# Autodesk Inventor assembly: Odom_Assembly_II
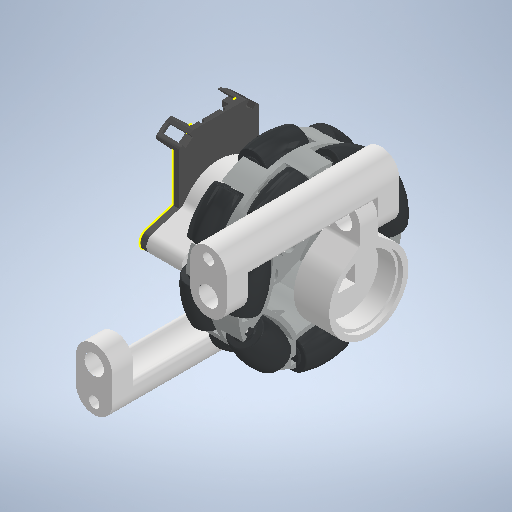
[picture p0: Inventor's stored thumbnail of the model, 512x512]
Saved by Autodesk Inventor 2025.1 (Build 291241020, 241B)
## iProperties
Created: 2024-11-16
Part Number: Odom_Assembly_II
Document SubType Name: Assembly
Designer: AtuStem
Author: AtuStem
## Documents named in this file (6)
- C:\Users\AtuStem\Documents\GitHub\ATUM-V5RC-High-Stakes-CAD\Protobot\Odom_Assembly_II.iam
- C:\Users\AtuStem\Documents\GitHub\ATUM-V5RC-High-Stakes-CAD\Protobot\Odom_Part1_Encoder_II.ipt
- C:\Users\AtuStem\Documents\GitHub\ATUM-V5RC-High-Stakes-CAD\Protobot\Odom_Part1_II.ipt
- C:\Users\AtuStem\Documents\GitHub\ATUM-V5RC-High-Stakes-CAD\Protobot\Encoder_Base.ipt
- C:\Users\AtuStem\Documents\GitHub\ATUM-V5RC-High-Stakes-CAD\Odometer_Test_Bracket.ipt
- C:\Users\AtuStem\Documents\GitHub\ATUM-V5RC-High-Stakes-CAD\Protobot\IQ_OMNI.iam
## Components (6 placed, 5 different names)
1. Odometer_Test_Bracket:1 — Mate:5, Mate:6, Flush:1
2. Odometer_Test_Bracket:2 — Mate:3, Mate:4, Flush:1
3. Odom_Part1_Encoder_II:1 — Mate:3, Mate:4, Mate:7, Mate:8, Mate:9, Mate:10, Mate:11
4. Odom_Part1_II:1 — Mate:5, Mate:6, Mate:7
5. IQ_OMNI:1 [sub-assembly] — Mate:8
6. Encoder_Base:1 — Mate:9, Mate:10, Mate:11
## Relationships (10: Mate 9, Flush 1)
- Mate:3: Odometer_Test_Bracket:2 ↔ Odom_Part1_Encoder_II:1
- Mate:4: Odometer_Test_Bracket:2 ↔ Odom_Part1_Encoder_II:1
- Mate:5: Odometer_Test_Bracket:1 ↔ Odom_Part1_II:1
- Mate:6: Odometer_Test_Bracket:1 ↔ Odom_Part1_II:1
- Flush:1: Odometer_Test_Bracket:1 ↔ Odometer_Test_Bracket:2
- Mate:7: Odom_Part1_Encoder_II:1 ↔ Odom_Part1_II:1
- Mate:8: Odom_Part1_Encoder_II:1 ↔ IQ_OMNI:1
- Mate:9: Odom_Part1_Encoder_II:1 ↔ Encoder_Base:1
- Mate:10: Odom_Part1_Encoder_II:1 ↔ Encoder_Base:1
- Mate:11: Odom_Part1_Encoder_II:1 ↔ Encoder_Base:1
